# Autodesk Inventor assembly: MotionBaseRough
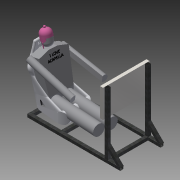
[picture p0: Inventor's stored thumbnail of the model, 180x180]
Saved by Autodesk Inventor 2015 SP1 (Build 190203100, 203)
## iProperties
Created: 2016-02-03
Part Number: MotionBaseRough
Document SubType Name: Assembly
Designer: guillemd
Mass: 152242 g
Surface Area: 81931.5 cm^2
Volume: 161529 cm^3
Density: 0.942511 g/cm^3
Author: guillemd
## Documents named in this file (8)
- C:\Users\guillemd\Desktop\Motion Base Rough model\MotionBaseRough.iam
- C:\Users\guillemd\Desktop\Motion Base Rough model\60_inch_square.ipt
- C:\Users\guillemd\Desktop\Motion Base Rough model\24_inch_square.ipt
- C:\Users\guillemd\Desktop\Motion Base Rough model\siege.ipt
- C:\Users\guillemd\Desktop\Motion Base Rough model\David_Mac_Jones.iam
- C:\Users\guillemd\Desktop\Motion Base Rough model\45degree_brace.ipt
- C:\Users\guillemd\Desktop\Motion Base Rough model\48_Inch_square.ipt
- C:\Users\guillemd\Desktop\Motion Base Rough model\Television.ipt
## Components (12 placed, 7 different names)
1. 60_inch_square:1 — Mate:1, Flush:1, Mate:3, Mate:4, Flush:2, Mate:13, Flush:12, Mate:14, Flush:13
2. 60_inch_square:2 — Mate:2, Flush:1, Mate:3, Flush:3, Flush:4, Flush:5, Mate:5, Mate:6, Mate:7, Flush:6, Flush:7, Mate:9, Mate:12, Flush:11, Mate:16, Flush:14
3. 24_inch_square:1 — Flush:3, Mate:5, Flush:6, Mate:8, Mate:10
4. 24_inch_square:2 — Flush:4, Mate:6, Mate:8
5. 24_inch_square:3 — Flush:5, Mate:7, Flush:7, Flush:9, Flush:10
6. siege:1 — Flush:8, Mate:9, Mate:10, Mate:11
7. David_Mac_Jones:1 [sub-assembly] — Mate:11
8. 45degree_brace:1 — Mate:16, Flush:14, Mate:17
9. 45degree_brace:2 — Mate:14, Flush:13, Mate:15
10. 48_Inch_square:1 — Mate:13, Flush:9, Flush:12, Mate:15, Mate:18
11. 48_Inch_square:2 — Mate:12, Flush:10, Flush:11, Mate:17, Flush:15, Flush:16
12. Television:1 — Mate:18, Flush:15, Flush:16
## Relationships (34: Mate 18, Flush 16)
- Mate:1: 60_inch_square:1
- Mate:2: 60_inch_square:2
- Flush:1: 60_inch_square:1 ↔ 60_inch_square:2
- Mate:3 (609.6 mm): 60_inch_square:1 ↔ 60_inch_square:2
- Mate:4 (304.8 mm): 60_inch_square:1
- Flush:2 (-762 mm): 60_inch_square:1
- Flush:3: 60_inch_square:2 ↔ 24_inch_square:1
- Flush:4: 60_inch_square:2 ↔ 24_inch_square:2
- Flush:5: 60_inch_square:2 ↔ 24_inch_square:3
- Mate:5: 60_inch_square:2 ↔ 24_inch_square:1
- Mate:6: 60_inch_square:2 ↔ 24_inch_square:2
- Mate:7: 60_inch_square:2 ↔ 24_inch_square:3
- Flush:6: 60_inch_square:2 ↔ 24_inch_square:1
- Mate:8 (457.2 mm): 24_inch_square:1 ↔ 24_inch_square:2
- Flush:7 (203.2 mm): 60_inch_square:2 ↔ 24_inch_square:3
- Flush:8: siege:1
- Mate:9: 60_inch_square:2 ↔ siege:1
- Mate:10: 24_inch_square:1 ↔ siege:1
- Mate:11: siege:1 ↔ David_Mac_Jones:1
- Mate:12: 60_inch_square:2 ↔ 48_Inch_square:2
- Mate:13: 60_inch_square:1 ↔ 48_Inch_square:1
- Flush:9: 24_inch_square:3 ↔ 48_Inch_square:1
- Flush:10: 24_inch_square:3 ↔ 48_Inch_square:2
- Flush:11: 60_inch_square:2 ↔ 48_Inch_square:2
- Flush:12: 60_inch_square:1 ↔ 48_Inch_square:1
- Mate:14: 60_inch_square:1 ↔ 45degree_brace:2
- Flush:13: 60_inch_square:1 ↔ 45degree_brace:2
- Mate:15: 45degree_brace:2 ↔ 48_Inch_square:1
- Mate:16: 60_inch_square:2 ↔ 45degree_brace:1
- Flush:14: 60_inch_square:2 ↔ 45degree_brace:1
- Mate:17: 45degree_brace:1 ↔ 48_Inch_square:2
- Mate:18: 48_Inch_square:1 ↔ Television:1
- Flush:15 (25.4 mm): 48_Inch_square:2 ↔ Television:1
- Flush:16: 48_Inch_square:2 ↔ Television:1
